# Autodesk Inventor assembly: Arduino UNO R3 and Screw shield v2
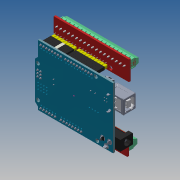
[picture p0: Inventor's stored thumbnail of the model, 180x180]
Saved by Autodesk Inventor 2017 SP1 (Build 210196100, 196)
## iProperties
Created: 2022-11-04
Part Number: Arduino UNO R3 and Screw shield v2
Document SubType Name: Assembly
Designer: Antonio
Author: Antonio
## Documents named in this file (4)
- C:\Users\Antonio\Documents\Inventor\Secador v2\Arduino UNO R3 screw shield v2\Arduino UNO R3 and Screw shield v2.iam
- C:\Users\Antonio\Documents\Inventor\Secador v2\Arduino Guapo.ipt
- C:\Users\Antonio\Documents\Inventor\Secador v2\Arduino UNO R3 screw shield v2\Arduino UNO R3 screw shield v2  Right.ipt
- C:\Users\Antonio\Documents\Inventor\Secador v2\Arduino UNO R3 screw shield v2\Arduino UNO R3 screw shield v2  Left.ipt
## Components (3 placed, 3 different names)
1. Arduino Guapo:1 — Coincidencia:3, Nivelación:1, Nivelación:2, Coincidencia:4, Nivelación:3, Nivelación:4
2. Arduino UNO R3 screw shield v2  Right:1 — Coincidencia:3, Nivelación:1, Nivelación:2
3. Arduino UNO R3 screw shield v2  Left:1 — Coincidencia:4, Nivelación:3, Nivelación:4
## Relationships (6: Flush 4, Mate 2)
- Coincidencia:3 [Mate]: Arduino Guapo:1 ↔ Arduino UNO R3 screw shield v2  Right:1
- Nivelación:1 [Flush]: Arduino Guapo:1 ↔ Arduino UNO R3 screw shield v2  Right:1
- Nivelación:2 [Flush]: Arduino Guapo:1 ↔ Arduino UNO R3 screw shield v2  Right:1
- Coincidencia:4 [Mate]: Arduino Guapo:1 ↔ Arduino UNO R3 screw shield v2  Left:1
- Nivelación:3 [Flush]: Arduino Guapo:1 ↔ Arduino UNO R3 screw shield v2  Left:1
- Nivelación:4 [Flush]: Arduino Guapo:1 ↔ Arduino UNO R3 screw shield v2  Left:1
